# Autodesk Inventor assembly: Actuator 1.6
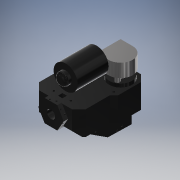
[picture p0: Inventor's stored thumbnail of the model, 180x180]
Saved by Autodesk Inventor 2017 SP1 (Build 210196100, 196)
## iProperties
Created: 2019-09-19
Part Number: Actuator 1.6
Document SubType Name: Assembly
Designer: Dell
Author: Dell
## Documents named in this file (15)
- C:\Users\Zach\Documents\GitHub\tr2\Actuator 2.0\Actuator 2.0.iam
- C:\Users\Zach\Documents\GitHub\tr2\Actuator 2.0\AC01.ipt
- C:\Users\Zach\Documents\GitHub\tr2\Actuator 2.0\AC02.ipt
- C:\Users\Zach\Documents\GitHub\tr2\Actuator 2.0\AC03.ipt
- C:\Users\Zach\Documents\GitHub\tr2\Actuator 2.0\AC05.ipt
- C:\Users\Zach\Documents\GitHub\tr2\Actuator 2.0\Slewing.iam
- C:\Users\Zach\Documents\GitHub\tr2\Actuator 2.0\Slip Ring.ipt
- C:\Users\Zach\Documents\GitHub\tr2\Actuator 2.0\8mm Mounting Hub.ipt
- C:\Users\Zach\Documents\GitHub\tr2\Actuator 2.0\AEAT-6012.ipt
- C:\Users\Zach\Documents\GitHub\tr2\Actuator 2.0\AC07.ipt
- C:\Users\Zach\Documents\GitHub\tr2\Actuator 2.0\Series Elastic Gearbox 1.2\Series Elastic Gearbox 1.2.iam
- C:\Users\Zach\OneDrive - slaterobots.com\STL\TS-40GZ7090.ipt
- C:\Users\Zach\Documents\GitHub\tr2\Actuator 2.0\Actuator 2.0\Design Accelerator\Spur Gears3.iam
- C:\Users\Zach\Documents\GitHub\tr2\Actuator 2.0\Actuator 2.0\Design Accelerator\Spur Gears4.iam
- C:\Users\Zach\Documents\GitHub\tr2\Actuator 2.0\Actuator 2.0\Design Accelerator\Spur Gears5.iam
## Components (16 placed, 12 different names)
1. AC01:1 — Mate:3, Mate:4, Mate:5, Mate:9, Mate:139, Mate:140, Mate:141, Mate:142
2. AC02:1 — Mate:9, Mate:16, Mate:70, Mate:71, Mate:77, Mate:78, Mate:112, Mate:121, Mate:122, Mate:135, Mate:136, Mate:137, Mate:138, Mate:139, Mate:140, Mate:141, Mate:142
3. AC03:1 — Mate:16
4. AC05:1 — Mate:6, Mate:7, Mate:8, Mate:23, Mate:24, Mate:25, Mate:90, Mate:91, Mate:92
5. Slewing:1 [sub-assembly] — Mate:3, Mate:4, Mate:5, Mate:6, Mate:7, Mate:8
6. Slip Ring:2 — Mate:23, Mate:24, Mate:25
7. 8mm Mounting Hub:1 — Mate:117, Mate:118, Mate:119
8. AEAT-6012:1 — Mate:80, Mate:88, Mate:124, Mate:132
9. AEAT-6012:2 — Mate:74, Mate:89, Mate:123, Mate:129
10. AC07:1 — Mate:70, Mate:71, Mate:74, Mate:89, Mate:122, Mate:123
11. AC07:2 — Mate:77, Mate:78, Mate:80, Mate:88, Mate:121, Mate:124
12. Series Elastic Gearbox 1.2:1 [sub-assembly] — Mate:90, Mate:91, Mate:92, Mate:113, Mate:114, Mate:116, Mate:120, Mate:130, Mate:131, Mate:133, Mate:134, Mate:135
13. TS-40GZ7090:1 — Mate:112, Mate:115, Mate:117, Mate:136, Mate:137, Mate:138
14. Spur Gears:1 [sub-assembly] — Mate:113, Mate:114, Mate:115, Mate:116, Mate:118, Mate:119, Mate:120, Flush:1, Rotation:1
15. Spur Gears:2 [sub-assembly] — Mate:130, Mate:131, Mate:132, Mate:133, Mate:134
16. Spur Gears:3 [sub-assembly] — Mate:129, Flush:1, Rotation:1
## Relationships (51: Mate 49, Flush 1, RelateRotation 1)
- Mate:3: AC01:1 ↔ Slewing:1
- Mate:4: AC01:1 ↔ Slewing:1
- Mate:5: AC01:1 ↔ Slewing:1
- Mate:6: AC05:1 ↔ Slewing:1
- Mate:7: AC05:1 ↔ Slewing:1
- Mate:8: AC05:1 ↔ Slewing:1
- Mate:9: AC01:1 ↔ AC02:1
- Mate:16: AC02:1 ↔ AC03:1
- Mate:23: AC05:1 ↔ Slip Ring:2
- Mate:24 (5 mm): AC05:1 ↔ Slip Ring:2
- Mate:25: AC05:1 ↔ Slip Ring:2
- Mate:70: AC02:1 ↔ AC07:1
- Mate:71: AC02:1 ↔ AC07:1
- Mate:74: AEAT-6012:2 ↔ AC07:1
- Mate:77: AC02:1 ↔ AC07:2
- Mate:78: AC02:1 ↔ AC07:2
- Mate:80: AEAT-6012:1 ↔ AC07:2
- Mate:88: AEAT-6012:1 ↔ AC07:2
- Mate:89: AEAT-6012:2 ↔ AC07:1
- Mate:90: AC05:1 ↔ Series Elastic Gearbox 1.2:1
- Mate:91: AC05:1 ↔ Series Elastic Gearbox 1.2:1
- Mate:92: AC05:1 ↔ Series Elastic Gearbox 1.2:1
- Mate:112: AC02:1 ↔ TS-40GZ7090:1
- Mate:113: Series Elastic Gearbox 1.2:1 ↔ Spur Gears:1
- Mate:114: Series Elastic Gearbox 1.2:1 ↔ Spur Gears:1
- Mate:115: TS-40GZ7090:1 ↔ Spur Gears:1
- Mate:116: Series Elastic Gearbox 1.2:1 ↔ Spur Gears:1
- Mate:117: 8mm Mounting Hub:1 ↔ TS-40GZ7090:1
- Mate:118: 8mm Mounting Hub:1 ↔ Spur Gears:1
- Mate:119: 8mm Mounting Hub:1 ↔ Spur Gears:1
- Mate:120: Series Elastic Gearbox 1.2:1 ↔ Spur Gears:1
- Mate:121: AC02:1 ↔ AC07:2
- Mate:122: AC02:1 ↔ AC07:1
- Mate:123: AEAT-6012:2 ↔ AC07:1
- Mate:124: AEAT-6012:1 ↔ AC07:2
- Mate:129: AEAT-6012:2 ↔ Spur Gears:3
- Flush:1: Spur Gears:1 ↔ Spur Gears:3
- Rotation:1 [RelateRotation] (1 ul): Spur Gears:1 ↔ Spur Gears:3
- Mate:130: Series Elastic Gearbox 1.2:1 ↔ Spur Gears:2
- Mate:131: Series Elastic Gearbox 1.2:1 ↔ Spur Gears:2
- Mate:132: AEAT-6012:1 ↔ Spur Gears:2
- Mate:133: Series Elastic Gearbox 1.2:1 ↔ Spur Gears:2
- Mate:134: Series Elastic Gearbox 1.2:1 ↔ Spur Gears:2
- Mate:135: AC02:1 ↔ Series Elastic Gearbox 1.2:1
- Mate:136: AC02:1 ↔ TS-40GZ7090:1
- Mate:137: AC02:1 ↔ TS-40GZ7090:1
- Mate:138: AC02:1 ↔ TS-40GZ7090:1
- Mate:139: AC01:1 ↔ AC02:1
- Mate:140: AC01:1 ↔ AC02:1
- Mate:141: AC01:1 ↔ AC02:1
- Mate:142: AC01:1 ↔ AC02:1
